# Autodesk Inventor assembly: sailAssembly
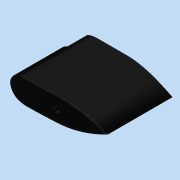
[picture p0: Inventor's stored thumbnail of the model, 180x180]
Saved by Autodesk Inventor 2017 (Build 210142000, 142)
## iProperties
Created: 2016-12-18
Part Number: sailAssembly
Document SubType Name: Assembly
Designer: techn
Author: techn
## Documents named in this file (4)
- D:\OneDrive\Documents\Other Projects\Submarine\CAD\midships\Sail\sailAssembly.iam
- D:\OneDrive\Documents\Other Projects\Submarine\CAD\midships\Sail\sailUpperPart1.ipt
- D:\OneDrive\Documents\Other Projects\Submarine\CAD\midships\Sail\sailUpperPart2.ipt
- D:\OneDrive\Documents\Other Projects\Submarine\CAD\midships\Sail\sailBottom.ipt
## Components (3 placed, 3 different names)
1. sailUpperPart1:1 — Mate:1, Mate:2, Mate:3, Mate:4
2. sailUpperPart2:1 — Mate:1, Mate:2, Mate:3, Flush:1, Mate:5
3. sailBottom:1 — Mate:4, Flush:1, Mate:5
## Relationships (6: Mate 5, Flush 1)
- Mate:1: sailUpperPart1:1 ↔ sailUpperPart2:1
- Mate:2: sailUpperPart1:1 ↔ sailUpperPart2:1
- Mate:3: sailUpperPart1:1 ↔ sailUpperPart2:1
- Mate:4: sailUpperPart1:1 ↔ sailBottom:1
- Flush:1: sailUpperPart2:1 ↔ sailBottom:1
- Mate:5: sailUpperPart2:1 ↔ sailBottom:1
